# Autodesk Inventor assembly: SensohalterMount
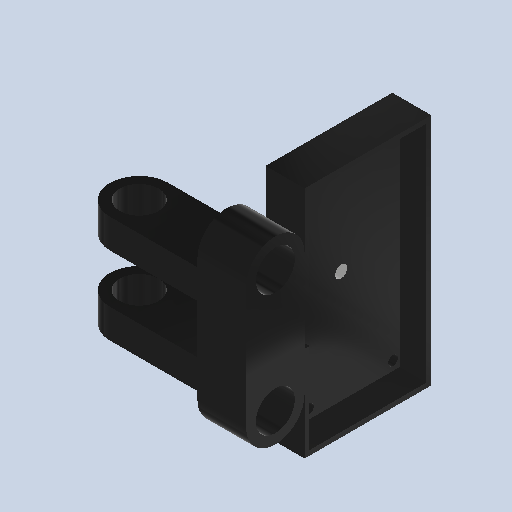
[picture p0: Inventor's stored thumbnail of the model, 512x512]
Saved by Autodesk Inventor 2023 (Build 270158000, 158)
## iProperties
Created: 2024-01-26
Part Number: SensohalterMount
Document SubType Name: Assembly
Designer: phili
Author: phili
## Documents named in this file (3)
- C:\Users\phili\FAUbox\Philipp\Bauprojekte\Ball_On_Beam\CAD\Bauteile\SensohalterMount.iam
- C:\Users\phili\FAUbox\Philipp\Bauprojekte\Ball_On_Beam\CAD\Bauteile\SensorHalter.ipt
- C:\Users\phili\FAUbox\Philipp\Bauprojekte\Ball_On_Beam\CAD\Bauteile\ObenMotor.ipt
## Components (2 placed, 2 different names)
1. SensorHalter:1 — Fluchtend:1, Passend:2, Passend:3
2. ObenMotor:1 — Fluchtend:1, Passend:2, Passend:3
## Relationships (3: Mate 2, Flush 1)
- Fluchtend:1 [Flush]: SensorHalter:1 ↔ ObenMotor:1
- Passend:2 [Mate] (-11.5 mm): SensorHalter:1 ↔ ObenMotor:1
- Passend:3 [Mate]: SensorHalter:1 ↔ ObenMotor:1
